# Autodesk Inventor assembly: Leg_Link_Flame_8
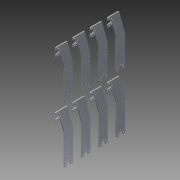
[picture p0: Inventor's stored thumbnail of the model, 180x180]
Saved by Autodesk Inventor 2013 (Build 170138000, 138)
## iProperties
Created: 2014-04-26
Part Number: Leg_Link_Flame_8
Document SubType Name: Assembly
Designer: andou
Author: andou
## Documents named in this file (2)
- C:\Users\andou\Documents\Inventor\RoboticsProject\project_4\Robot\Leg_Link_Flame_8.iam
- C:\Users\andou\Documents\Inventor\RoboticsProject\project_4\Robot\Leg_Link_Flame.ipt
## Components (8 placed, 1 different names)
1. Leg_Link_Flame:1
2. Leg_Link_Flame:2
3. Leg_Link_Flame:3
4. Leg_Link_Flame:4
5. Leg_Link_Flame:5
6. Leg_Link_Flame:6
7. Leg_Link_Flame:7
8. Leg_Link_Flame:8
## Component patterns: (8 elements, first: Leg_Link_Flame:1)
